# Autodesk Inventor assembly: ES Battery 3 Cell
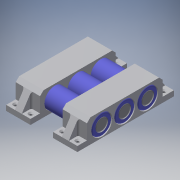
[picture p0: Inventor's stored thumbnail of the model, 180x180]
Saved by Autodesk Inventor 2016 SP1 (Build 200210100, 210)
## iProperties
Created: 2016-12-17
Part Number: ES Battery 3 Cell
Document SubType Name: Assembly
Designer: eschr_000
Author: eschr_000
## Documents named in this file (3)
- C:\Users\eschr_000\Documents\School\Hermes\CAD\CADD\ES Battery 3 Cell.iam
- C:\Users\eschr_000\Documents\School\Hermes\CAD\CADD\Battery_Mount_1U_Hermes_V1.ipt
- C:\Users\eschr_000\Documents\School\Hermes\CAD\CADD\18650_thmjpr.ipt
## Components (5 placed, 2 different names)
1. Battery_Mount_1U_Hermes_V1:1 — Mate:1, Mate:2, Mate:3, Flush:1, Flush:2, Flush:3
2. 18650_thmjpr:1 — Mate:3, Flush:1, Mate:4, Flush:4
3. 18650_thmjpr:2 — Mate:2, Flush:2
4. 18650_thmjpr:3 — Mate:1, Flush:3, Mate:5
5. Battery_Mount_1U_Hermes_V1:2 — Mate:4, Mate:5, Flush:4
## Relationships (9: Mate 5, Flush 4)
- Mate:1: Battery_Mount_1U_Hermes_V1:1 ↔ 18650_thmjpr:3
- Mate:2: Battery_Mount_1U_Hermes_V1:1 ↔ 18650_thmjpr:2
- Mate:3: Battery_Mount_1U_Hermes_V1:1 ↔ 18650_thmjpr:1
- Flush:1: Battery_Mount_1U_Hermes_V1:1 ↔ 18650_thmjpr:1
- Flush:2: Battery_Mount_1U_Hermes_V1:1 ↔ 18650_thmjpr:2
- Flush:3: Battery_Mount_1U_Hermes_V1:1 ↔ 18650_thmjpr:3
- Mate:4: 18650_thmjpr:1 ↔ Battery_Mount_1U_Hermes_V1:2
- Mate:5: 18650_thmjpr:3 ↔ Battery_Mount_1U_Hermes_V1:2
- Flush:4: 18650_thmjpr:1 ↔ Battery_Mount_1U_Hermes_V1:2
